# Autodesk Inventor assembly: Hinge and Leaf Assembly
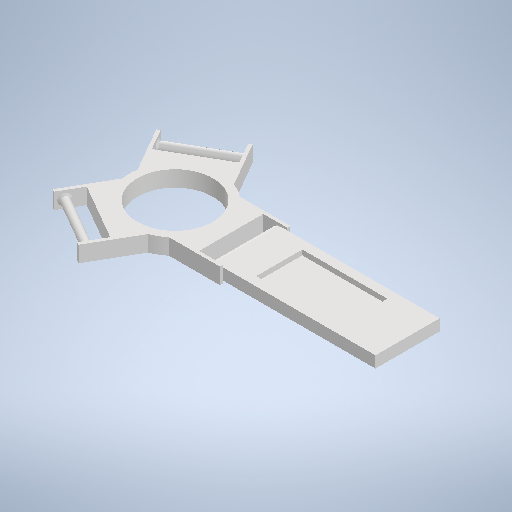
[picture p0: Inventor's stored thumbnail of the model, 512x512]
Saved by Autodesk Inventor 2025 (Build 290162000, 162)
## iProperties
Created: 2024-06-14
Part Number: Hinge and Leaf Assembly
Document SubType Name: Assembly
Designer: track
Author: track
## Documents named in this file (3)
- C:\Users\track\OneDrive\Documents\Hinge and Leaf Assembly.iam
- C:\Users\track\OneDrive\Documents\Connector and Hidnges.ipt
- C:\Users\track\OneDrive\Documents\Leaf.ipt
## Components (2 placed, 2 different names)
1. Connector and Hidnges:1 — Cylindrical:1, Rotational:1
2. Leaf:1 — Cylindrical:1, Rotational:1
## Relationships (2: CylindricalJoint 1, RevoluteJoint 1)
- Cylindrical:1: Connector and Hidnges:1 ↔ Leaf:1
- Rotational:1 [RevoluteJoint]: Connector and Hidnges:1 ↔ Leaf:1
